# Autodesk Inventor assembly: Montiert
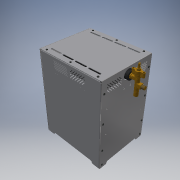
[picture p0: Inventor's stored thumbnail of the model, 180x180]
Saved by Autodesk Inventor 2018 (Build 220112000, 112)
## iProperties
Created: 2017-11-12
Part Number: Montiert
Material: Generisch
Document SubType Name: Assembly
## Documents named in this file (21)
- C:\git\RoKu-ProjectX01\Konstruktion\Montiert.iam
- C:\git\RoKu-ProjectX01\Konstruktion\Brenner.ipt
- C:\git\RoKu-ProjectX01\Konstruktion\Gegenhalter.ipt
- C:\git\RoKu-ProjectX01\Konstruktion\BrennerBrennTeil.ipt
- C:\git\RoKu-ProjectX01\Konstruktion\Back.ipt
- C:\git\RoKu-ProjectX01\Konstruktion\Seite.ipt
- C:\git\RoKu-ProjectX01\Konstruktion\Front.ipt
- C:\git\RoKu-ProjectX01\Konstruktion\Deckel.ipt
- C:\git\RoKu-ProjectX01\Konstruktion\BrennerHalter.ipt
- C:\Users\kuckal\Documents\Inventor\Content Center Files\R2018\de-DE\ISO 7380-1\ISO 7380-1 - M4 x 8.ipt
- C:\Users\kuckal\Documents\Inventor\Content Center Files\R2018\de-DE\ISO 7380-1\ISO 7380-1 - M4 x 6.ipt
- C:\Users\kuckal\Documents\Inventor\Content Center Files\R2018\de-DE\DIN EN 24 036(2)\DIN EN 24 036 - M4.ipt
- C:\git\RoKu-ProjectX01\Konstruktion\Boden.ipt
- C:\Users\kuckal\Documents\Inventor\Content Center Files\R2018\de-DE\DIN 433-1  A\DIN 433 - 4,3.ipt
- C:\Users\kuckal\Documents\Inventor\Content Center Files\R2018\de-DE\DIN 9021\DIN 9021 - 4,3.ipt
- C:\Users\kuckal\Documents\Inventor\Content Center Files\R2018\de-DE\ISO 7380-1\ISO 7380-1 - M4 x 10.ipt
- C:\git\RoKu-ProjectX01\Konstruktion\Rost_Beef.ipt
- C:\git\RoKu-ProjectX01\Konstruktion\Rost_Burgee.ipt
- C:\git\RoKu-ProjectX01\Konstruktion\Rost_Heber.ipt
- C:\git\RoKu-ProjectX01\Konstruktion\Gasanschluss.ipt
- C:\git\RoKu-ProjectX01\Konstruktion\Einschub.ipt
## Components (96 placed, 20 different names)
1. Brenner:1 — Fluchtend:1, Fluchtend:2, Fluchtend:3, Passend:1, Passend:2, Fluchtend:4, Passend:4, Fluchtend:13, Fluchtend:14, Einfügen:37, Einfügen:38, Einfügen:39, Einfügen:40, Einfügen:41, Einfügen:42, Einfügen:43, Einfügen:44, Einfügen:45, Einfügen:46, Einfügen:47, Einfügen:48, Passend:13, Passend:24, Passend:25
2. Gegenhalter:1 — Passend:1, Passend:2, Einfügen:55, Einfügen:56, Einfügen:57, Einfügen:58, Einfügen:59, Einfügen:60, Einfügen:61, Einfügen:62, Einfügen:63, Einfügen:64, Einfügen:65, Einfügen:66, Passend:20
3. BrennerBrennTeil:1 — Fluchtend:4
4. Back:1 — Passend:4, Passend:5, Passend:6, Fluchtend:6, Fluchtend:7, Passend:7, Fluchtend:8, Fluchtend:9, Einfügen:25, Einfügen:26, Einfügen:27, Einfügen:28, Einfügen:29, Einfügen:30, Fluchtend:15, Einfügen:69, Einfügen:70, Passend:13, Passend:14, Passend:17, Fluchtend:18
5. Seite:1 — Passend:6, Fluchtend:6, Fluchtend:7, Passend:8, Fluchtend:11, Passend:9, Fluchtend:12, Einfügen:52, Einfügen:53, Einfügen:54, Passend:12, Einfügen:83, Einfügen:88
6. Seite:2 — Passend:7, Fluchtend:8, Fluchtend:9, Fluchtend:10, Einfügen:49, Einfügen:50, Einfügen:51, Passend:11, Einfügen:71, Einfügen:78
7. Front:1 — Passend:8, Fluchtend:10, Fluchtend:11, Passend:10, Einfügen:15, Einfügen:16, Einfügen:17, Einfügen:18, Einfügen:19, Einfügen:20, Einfügen:67, Einfügen:68, Fluchtend:17, Fluchtend:20, Passend:27, Passend:28
8. Deckel:1 — Passend:9, Fluchtend:12, Passend:10, Einfügen:31, Einfügen:32, Einfügen:33, Einfügen:34, Einfügen:35, Einfügen:36
9. BrennerHalter:1 — Fluchtend:13, Fluchtend:14
10. Boden:1 — Fluchtend:15, Passend:11, Passend:12, Passend:16
11. Rost_Beef:1 — Passend:14, Passend:15, Passend:16, Passend:19, Passend:21, Passend:22, Passend:23
12. Rost_Burgee:1 — Passend:17, Passend:18, Passend:19, Passend:20, Fluchtend:19
13. Rost_Heber:1 — Passend:21, Passend:22, Passend:23
14. Gasanschluss:1 — Passend:24, Fluchtend:16, Passend:25
15. Einschub:3 — Fluchtend:20, Fluchtend:21
16. Einschub:2 — Passend:26, Passend:27, Passend:28
17. ISO 7380-1 M4 x 6:15 — Einfügen:15
18. ISO 7380-1 M4 x 6:16 — Einfügen:16
19. ISO 7380-1 M4 x 6:17 — Einfügen:17
20. ISO 7380-1 M4 x 6:18 — Einfügen:18
21. ISO 7380-1 M4 x 6:19 — Einfügen:19
22. ISO 7380-1 M4 x 6:20 — Einfügen:20
23. ISO 7380-1 M4 x 8:1 — Einfügen:25
24. ISO 7380-1 M4 x 8:2 — Einfügen:26
25. ISO 7380-1 M4 x 8:3 — Einfügen:27
26. ISO 7380-1 M4 x 8:4 — Einfügen:28
27. ISO 7380-1 M4 x 8:5 — Einfügen:29
28. ISO 7380-1 M4 x 8:6 — Einfügen:30
29. ISO 7380-1 M4 x 8:7 — Einfügen:31
30. ISO 7380-1 M4 x 8:8 — Einfügen:32
31. ISO 7380-1 M4 x 8:9 — Einfügen:33
32. ISO 7380-1 M4 x 8:10 — Einfügen:34
33. ISO 7380-1 M4 x 8:11 — Einfügen:35
34. ISO 7380-1 M4 x 8:12 — Einfügen:36
35. ISO 7380-1 M4 x 8:13 — Einfügen:37
36. ISO 7380-1 M4 x 8:14 — Einfügen:38
37. ISO 7380-1 M4 x 8:15 — Einfügen:39
38. ISO 7380-1 M4 x 8:16 — Einfügen:40
39. ISO 7380-1 M4 x 8:17 — Einfügen:41
40. ISO 7380-1 M4 x 8:18 — Einfügen:42
41. ISO 7380-1 M4 x 8:19 — Einfügen:43
42. ISO 7380-1 M4 x 8:20 — Einfügen:44
43. ISO 7380-1 M4 x 8:21 — Einfügen:45
44. ISO 7380-1 M4 x 8:22 — Einfügen:46
45. ISO 7380-1 M4 x 8:23 — Einfügen:47
46. ISO 7380-1 M4 x 8:24 — Einfügen:48
47. DIN EN 24036 M4:1 — Einfügen:49
48. DIN EN 24036 M4:2 — Einfügen:50
49. DIN EN 24036 M4:3 — Einfügen:51
50. DIN EN 24036 M4:4 — Einfügen:52
51. DIN EN 24036 M4:5 — Einfügen:53
52. DIN EN 24036 M4:6 — Einfügen:54
53. DIN EN 24036 M4:7 — Einfügen:55
54. DIN EN 24036 M4:8 — Einfügen:56
55. DIN EN 24036 M4:9 — Einfügen:57
56. DIN EN 24036 M4:10 — Einfügen:58
57. DIN EN 24036 M4:11 — Einfügen:59
58. DIN EN 24036 M4:12 — Einfügen:60
59. DIN EN 24036 M4:13 — Einfügen:61
60. DIN EN 24036 M4:14 — Einfügen:62
61. DIN EN 24036 M4:15 — Einfügen:63
62. DIN EN 24036 M4:16 — Einfügen:64
63. DIN EN 24036 M4:17 — Einfügen:65
64. DIN EN 24036 M4:18 — Einfügen:66
65. DIN 433-1 A 4,3:6 — Einfügen:78, Einfügen:79
66. DIN 433-1 A 4,3:7 — Einfügen:79, Einfügen:80
67. DIN 433-1 A 4,3:8 — Einfügen:80, Einfügen:81
68. DIN 433-1 A 4,3:9 — Einfügen:81, Einfügen:82
69. DIN 433-1 A 4,3:10 — Einfügen:82, Einfügen:95
70. DIN 433-1 A 4,3:11 — Einfügen:83, Einfügen:84
71. DIN 433-1 A 4,3:12 — Einfügen:84, Einfügen:85
72. DIN 433-1 A 4,3:13 — Einfügen:85, Einfügen:86
73. DIN 433-1 A 4,3:14 — Einfügen:86, Einfügen:87
74. DIN 433-1 A 4,3:15 — Einfügen:87, Einfügen:94
75. DIN 433-1 A 4,3:16 — Einfügen:88, Einfügen:89
76. DIN 433-1 A 4,3:17 — Einfügen:89, Einfügen:90
77. DIN 433-1 A 4,3:18 — Einfügen:90, Einfügen:91
78. DIN 433-1 A 4,3:19 — Einfügen:91, Einfügen:92
79. DIN 433-1 A 4,3:20 — Einfügen:92, Einfügen:93
80. DIN 9021 4,3:2 — Einfügen:93, Einfügen:98
81. DIN 9021 4,3:3 — Einfügen:94, Einfügen:97
82. DIN 9021 4,3:4 — Einfügen:95, Einfügen:96
83. DIN EN 24036 M4:20 — Einfügen:96
84. DIN EN 24036 M4:21 — Einfügen:97
85. DIN EN 24036 M4:22 — Einfügen:98
86. ISO 7380-1 M4 x 10:1 — Einfügen:67
87. ISO 7380-1 M4 x 10:2 — Einfügen:68
88. ISO 7380-1 M4 x 10:3 — Einfügen:69
89. ISO 7380-1 M4 x 10:4 — Einfügen:70
90. DIN 433-1 A 4,3:1 — Einfügen:71, Einfügen:72
91. DIN 433-1 A 4,3:2 — Einfügen:72, Einfügen:73
92. DIN 433-1 A 4,3:3 — Einfügen:73, Einfügen:74
93. DIN 433-1 A 4,3:4 — Einfügen:74, Einfügen:75
94. DIN 433-1 A 4,3:5 — Einfügen:75, Einfügen:76
95. DIN 9021 4,3:1 — Einfügen:76, Einfügen:77
96. DIN EN 24036 M4:19 — Einfügen:77
## Relationships (127: Insert 80, Mate 27, Flush 20)
- Fluchtend:1 [Flush]: Brenner:1
- Fluchtend:2 [Flush]: Brenner:1
- Fluchtend:3 [Flush]: Brenner:1
- Passend:1 [Mate] (2 mm): Brenner:1 ↔ Gegenhalter:1
- Passend:2 [Mate]: Brenner:1 ↔ Gegenhalter:1
- Fluchtend:4 [Flush]: Brenner:1 ↔ BrennerBrennTeil:1
- Passend:4 [Mate] (-12 mm): Brenner:1 ↔ Back:1
- Passend:5 [Mate]: Back:1
- Passend:6 [Mate]: Back:1 ↔ Seite:1
- Fluchtend:6 [Flush]: Back:1 ↔ Seite:1
- Fluchtend:7 [Flush]: Back:1 ↔ Seite:1
- Passend:7 [Mate]: Back:1 ↔ Seite:2
- Fluchtend:8 [Flush]: Back:1 ↔ Seite:2
- Fluchtend:9 [Flush]: Back:1 ↔ Seite:2
- Passend:8 [Mate]: Seite:1 ↔ Front:1
- Fluchtend:10 [Flush]: Seite:2 ↔ Front:1
- Fluchtend:11 [Flush]: Seite:1 ↔ Front:1
- Passend:9 [Mate]: Seite:1 ↔ Deckel:1
- Fluchtend:12 [Flush]: Seite:1 ↔ Deckel:1
- Passend:10 [Mate]: Front:1 ↔ Deckel:1
- Fluchtend:13 [Flush]: Brenner:1 ↔ BrennerHalter:1
- Fluchtend:14 [Flush]: Brenner:1 ↔ BrennerHalter:1
- Einfügen:15 [Insert]: Front:1 ↔ ISO 7380-1 M4 x 6:15
- Einfügen:16 [Insert]: Front:1 ↔ ISO 7380-1 M4 x 6:16
- Einfügen:17 [Insert]: Front:1 ↔ ISO 7380-1 M4 x 6:17
- Einfügen:18 [Insert]: Front:1 ↔ ISO 7380-1 M4 x 6:18
- Einfügen:19 [Insert]: Front:1 ↔ ISO 7380-1 M4 x 6:19
- Einfügen:20 [Insert]: Front:1 ↔ ISO 7380-1 M4 x 6:20
- Einfügen:25 [Insert]: Back:1 ↔ ISO 7380-1 M4 x 8:1
- Einfügen:26 [Insert]: Back:1 ↔ ISO 7380-1 M4 x 8:2
- Einfügen:27 [Insert]: Back:1 ↔ ISO 7380-1 M4 x 8:3
- Einfügen:28 [Insert]: Back:1 ↔ ISO 7380-1 M4 x 8:4
- Einfügen:29 [Insert]: Back:1 ↔ ISO 7380-1 M4 x 8:5
- Einfügen:30 [Insert]: Back:1 ↔ ISO 7380-1 M4 x 8:6
- Einfügen:31 [Insert]: Deckel:1 ↔ ISO 7380-1 M4 x 8:7
- Einfügen:32 [Insert]: Deckel:1 ↔ ISO 7380-1 M4 x 8:8
- Einfügen:33 [Insert]: Deckel:1 ↔ ISO 7380-1 M4 x 8:9
- Einfügen:34 [Insert]: Deckel:1 ↔ ISO 7380-1 M4 x 8:10
- Einfügen:35 [Insert]: Deckel:1 ↔ ISO 7380-1 M4 x 8:11
- Einfügen:36 [Insert]: Deckel:1 ↔ ISO 7380-1 M4 x 8:12
- Einfügen:37 [Insert]: Brenner:1 ↔ ISO 7380-1 M4 x 8:13
- Einfügen:38 [Insert]: Brenner:1 ↔ ISO 7380-1 M4 x 8:14
- Einfügen:39 [Insert]: Brenner:1 ↔ ISO 7380-1 M4 x 8:15
- Einfügen:40 [Insert]: Brenner:1 ↔ ISO 7380-1 M4 x 8:16
- Einfügen:41 [Insert]: Brenner:1 ↔ ISO 7380-1 M4 x 8:17
- Einfügen:42 [Insert]: Brenner:1 ↔ ISO 7380-1 M4 x 8:18
- Einfügen:43 [Insert]: Brenner:1 ↔ ISO 7380-1 M4 x 8:19
- Einfügen:44 [Insert]: Brenner:1 ↔ ISO 7380-1 M4 x 8:20
- Einfügen:45 [Insert]: Brenner:1 ↔ ISO 7380-1 M4 x 8:21
- Einfügen:46 [Insert]: Brenner:1 ↔ ISO 7380-1 M4 x 8:22
- Einfügen:47 [Insert]: Brenner:1 ↔ ISO 7380-1 M4 x 8:23
- Einfügen:48 [Insert]: Brenner:1 ↔ ISO 7380-1 M4 x 8:24
- Einfügen:49 [Insert]: Seite:2 ↔ DIN EN 24036 M4:1
- Einfügen:50 [Insert]: Seite:2 ↔ DIN EN 24036 M4:2
- Einfügen:51 [Insert]: Seite:2 ↔ DIN EN 24036 M4:3
- Einfügen:52 [Insert]: Seite:1 ↔ DIN EN 24036 M4:4
- Einfügen:53 [Insert]: Seite:1 ↔ DIN EN 24036 M4:5
- Einfügen:54 [Insert]: Seite:1 ↔ DIN EN 24036 M4:6
- Einfügen:55 [Insert]: Gegenhalter:1 ↔ DIN EN 24036 M4:7
- Einfügen:56 [Insert]: Gegenhalter:1 ↔ DIN EN 24036 M4:8
- Einfügen:57 [Insert]: Gegenhalter:1 ↔ DIN EN 24036 M4:9
- Einfügen:58 [Insert]: Gegenhalter:1 ↔ DIN EN 24036 M4:10
- Einfügen:59 [Insert]: Gegenhalter:1 ↔ DIN EN 24036 M4:11
- Einfügen:60 [Insert]: Gegenhalter:1 ↔ DIN EN 24036 M4:12
- Einfügen:61 [Insert]: Gegenhalter:1 ↔ DIN EN 24036 M4:13
- Einfügen:62 [Insert]: Gegenhalter:1 ↔ DIN EN 24036 M4:14
- Einfügen:63 [Insert]: Gegenhalter:1 ↔ DIN EN 24036 M4:15
- Einfügen:64 [Insert]: Gegenhalter:1 ↔ DIN EN 24036 M4:16
- Einfügen:65 [Insert]: Gegenhalter:1 ↔ DIN EN 24036 M4:17
- Einfügen:66 [Insert]: Gegenhalter:1 ↔ DIN EN 24036 M4:18
- Fluchtend:15 [Flush]: Back:1 ↔ Boden:1
- Passend:11 [Mate] (0.1 mm): Seite:2 ↔ Boden:1
- Passend:12 [Mate] (0.1 mm): Seite:1 ↔ Boden:1
- Einfügen:67 [Insert]: Front:1 ↔ ISO 7380-1 M4 x 10:1
- Einfügen:68 [Insert]: Front:1 ↔ ISO 7380-1 M4 x 10:2
- Einfügen:69 [Insert]: Back:1 ↔ ISO 7380-1 M4 x 10:3
- Einfügen:70 [Insert]: Back:1 ↔ ISO 7380-1 M4 x 10:4
- Einfügen:71 [Insert]: Seite:2 ↔ DIN 433-1 A 4,3:1
- Einfügen:72 [Insert]: DIN 433-1 A 4,3:1 ↔ DIN 433-1 A 4,3:2
- Einfügen:73 [Insert]: DIN 433-1 A 4,3:2 ↔ DIN 433-1 A 4,3:3
- Einfügen:74 [Insert]: DIN 433-1 A 4,3:3 ↔ DIN 433-1 A 4,3:4
- Einfügen:75 [Insert]: DIN 433-1 A 4,3:4 ↔ DIN 433-1 A 4,3:5
- Einfügen:76 [Insert]: DIN 433-1 A 4,3:5 ↔ DIN 9021 4,3:1
- Einfügen:77 [Insert]: DIN 9021 4,3:1 ↔ DIN EN 24036 M4:19
- Einfügen:78 [Insert]: Seite:2 ↔ DIN 433-1 A 4,3:6
- Einfügen:79 [Insert]: DIN 433-1 A 4,3:6 ↔ DIN 433-1 A 4,3:7
- Einfügen:80 [Insert]: DIN 433-1 A 4,3:7 ↔ DIN 433-1 A 4,3:8
- Einfügen:81 [Insert]: DIN 433-1 A 4,3:8 ↔ DIN 433-1 A 4,3:9
- Einfügen:82 [Insert]: DIN 433-1 A 4,3:9 ↔ DIN 433-1 A 4,3:10
- Einfügen:83 [Insert]: Seite:1 ↔ DIN 433-1 A 4,3:11
- Einfügen:84 [Insert]: DIN 433-1 A 4,3:11 ↔ DIN 433-1 A 4,3:12
- Einfügen:85 [Insert]: DIN 433-1 A 4,3:12 ↔ DIN 433-1 A 4,3:13
- Einfügen:86 [Insert]: DIN 433-1 A 4,3:13 ↔ DIN 433-1 A 4,3:14
- Einfügen:87 [Insert]: DIN 433-1 A 4,3:14 ↔ DIN 433-1 A 4,3:15
- Einfügen:88 [Insert]: Seite:1 ↔ DIN 433-1 A 4,3:16
- Einfügen:89 [Insert]: DIN 433-1 A 4,3:16 ↔ DIN 433-1 A 4,3:17
- Einfügen:90 [Insert]: DIN 433-1 A 4,3:17 ↔ DIN 433-1 A 4,3:18
- Einfügen:91 [Insert]: DIN 433-1 A 4,3:18 ↔ DIN 433-1 A 4,3:19
- Einfügen:92 [Insert]: DIN 433-1 A 4,3:19 ↔ DIN 433-1 A 4,3:20
- Einfügen:93 [Insert]: DIN 433-1 A 4,3:20 ↔ DIN 9021 4,3:2
- Einfügen:94 [Insert]: DIN 433-1 A 4,3:15 ↔ DIN 9021 4,3:3
- Einfügen:95 [Insert]: DIN 433-1 A 4,3:10 ↔ DIN 9021 4,3:4
- Einfügen:96 [Insert]: DIN 9021 4,3:4 ↔ DIN EN 24036 M4:20
- Einfügen:97 [Insert]: DIN 9021 4,3:3 ↔ DIN EN 24036 M4:21
- Einfügen:98 [Insert]: DIN 9021 4,3:2 ↔ DIN EN 24036 M4:22
- Passend:13 [Mate]: Brenner:1 ↔ Back:1
- Passend:14 [Mate]: Back:1 ↔ Rost_Beef:1
- Passend:15 [Mate]: Rost_Beef:1
- Passend:16 [Mate]: Boden:1 ↔ Rost_Beef:1
- Passend:17 [Mate]: Back:1 ↔ Rost_Burgee:1
- Passend:18 [Mate]: Rost_Burgee:1
- Passend:19 [Mate]: Rost_Beef:1 ↔ Rost_Burgee:1
- Passend:20 [Mate]: Gegenhalter:1 ↔ Rost_Burgee:1
- Passend:21 [Mate]: Rost_Beef:1 ↔ Rost_Heber:1
- Passend:22 [Mate] (2 mm): Rost_Beef:1 ↔ Rost_Heber:1
- Passend:23 [Mate]: Rost_Beef:1 ↔ Rost_Heber:1
- Passend:24 [Mate]: Brenner:1 ↔ Gasanschluss:1
- Fluchtend:16 [Flush]: Gasanschluss:1
- Passend:25 [Mate]: Brenner:1 ↔ Gasanschluss:1
- Fluchtend:17 [Flush] (10 mm): Front:1
- Fluchtend:18 [Flush] (10 mm): Back:1
- Fluchtend:19 [Flush] (-2 mm): Rost_Burgee:1
- Fluchtend:20 [Flush]: Front:1 ↔ Einschub:3
- Fluchtend:21 [Flush]: Einschub:3
- Passend:26 [Mate]: Einschub:2
- Passend:27 [Mate]: Front:1 ↔ Einschub:2
- Passend:28 [Mate]: Front:1 ↔ Einschub:2
